# Autodesk Inventor assembly: HUDSON-1-52
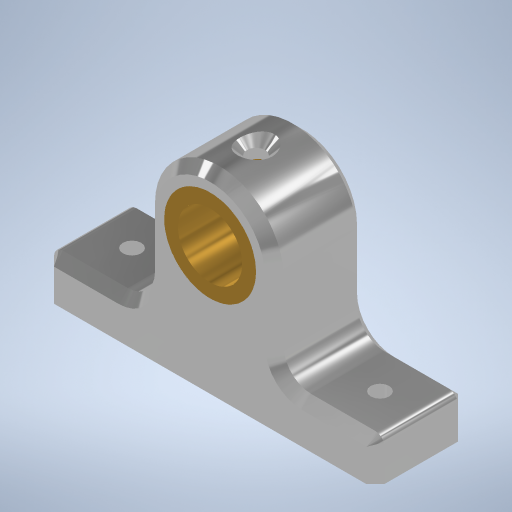
[picture p0: Inventor's stored thumbnail of the model, 512x512]
Saved by Autodesk Inventor 2024.2 (Build 282272000, 272)
## iProperties
Created: 2024-10-24
Part Number: HUDSON-1-52
Document SubType Name: Assembly
Designer: Precisión-05
Author: Precisión-05
## Documents named in this file (3)
- C:\Users\Precisión-05\Desktop\Nueva carpeta\HUDSON-1-52.iam
- C:\Users\Precisión-05\Desktop\Nueva carpeta\Part1.ipt
- C:\Users\Precisión-05\Desktop\Nueva carpeta\pt2.ipt
## Components (2 placed, 2 different names)
1. Part1:1 — Cylindrical:1
2. pt2:1 — Cylindrical:1
## Relationships (1: CylindricalJoint 1)
- Cylindrical:1: Part1:1 ↔ pt2:1
